# Autodesk Inventor assembly: Fr.wing_assy
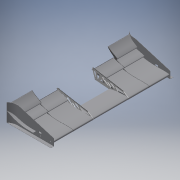
[picture p0: Inventor's stored thumbnail of the model, 180x180]
Saved by Autodesk Inventor 2018 (Build 220112000, 112)
## iProperties
Created: 2018-03-05
Part Number: Fr.wing_assy
Material: 一般
Document SubType Name: Assembly
Designer: ku_sk
Mass: 11232.8 g
Surface Area: 27769.7 cm^2
Volume: 11454.5 cm^3
Density: 0.980642 g/cm^3
Author: ku_sk
## Documents named in this file (19)
- Z:\各班フォルダ\2018\ボディ\エアロ\Aero\KS-15\Fr.wing\Fr.wing_assy.iam
- Z:\各班フォルダ\2018\ボディ\エアロ\Aero\KS-15\Fr.wing\parts\mainflap_side\mainflap_side.iam
- Z:\各班フォルダ\2018\ボディ\エアロ\Aero\KS-15\Fr.wing\parts\mainflap_center\mainflap_center.iam
- Z:\各班フォルダ\2018\ボディ\エアロ\Aero\KS-15\Fr.wing\parts\subflap\subflap.iam
- Z:\各班フォルダ\2018\ボディ\エアロ\Aero\KS-15\Fr.wing\parts\bracket1\bracket1.ipt
- Z:\各班フォルダ\2018\ボディ\エアロ\Aero\KS-15\Fr.wing\parts\bracket2.ipt
- Z:\各班フォルダ\2018\ボディ\エアロ\Aero\KS-15\Fr.wing\parts\axis_f3.ipt
- Z:\各班フォルダ\2018\ボディ\エアロ\Aero\KS-15\Fr.wing\parts\axis_f2.ipt
- Z:\各班フォルダ\2018\ボディ\エアロ\Aero\KS-15\Fr.wing\parts\axis_f1.ipt
- Z:\各班フォルダ\2018\ボディ\エアロ\Aero\KS-15\Fr.wing\parts\subflap_top.ipt
- Z:\各班フォルダ\2018\ボディ\エアロ\Aero\KS-15\Fr.wing\parts\subflap_top1.ipt
- Z:\各班フォルダ\2018\ボディ\エアロ\Aero\KS-15\Fr.wing\parts\gurnee.ipt
- Z:\各班フォルダ\2018\ボディ\エアロ\Aero\KS-15\Fr.wing\parts\gurnee_top.ipt
- Z:\各班フォルダ\2018\ボディ\エアロ\Aero\KS-15\Fr.wing\parts\endplate\ver.2\endplate_ver2.iam
- Z:\各班フォルダ\2018\ボディ\エアロ\Aero\KS-15\Fr.wing\parts\endplate\ver.2\endplate_ver21.iam
- Z:\各班フォルダ\2018\ボディ\エアロ\Aero\KS-15\Fr.wing\parts\splitter\splitter.iam
- Z:\各班フォルダ\2018\ボディ\エアロ\Aero\KS-15\Fr.wing\parts\splitter\splitter_MIR.iam
- Z:\各班フォルダ\2018\ボディ\エアロ\Aero\KS-15\Fr.wing\parts\collar_5.ipt
- Z:\各班フォルダ\2018\ボディ\エアロ\Aero\KS-15\Fr.wing\parts\collar_10.ipt
## Components (37 placed, 18 different names)
1. mainflap_center:1 [sub-assembly] — フラッシュ:1, メイト:1, メイト:4, メイト:5, メイト:6, メイト:7, 角度:1, メイト:50, メイト:51, メイト:52, メイト:53, メイト:54, メイト:55
2. mainflap_side:1 [sub-assembly] — メイト:4, メイト:7, メイト:8, メイト:9, メイト:10, フラッシュ:2, メイト:46, メイト:56, メイト:57, メイト:64
3. mainflap_side:2 [sub-assembly] — メイト:5, メイト:6, メイト:11, メイト:12, メイト:13, フラッシュ:4, メイト:49, メイト:65, メイト:93
4. mainflap_side:3 [sub-assembly] — メイト:8, メイト:9, メイト:10, フラッシュ:3, メイト:78, メイト:79, フラッシュ:20
5. mainflap_side:4 [sub-assembly] — メイト:11, メイト:12, メイト:13, フラッシュ:5
6. subflap:1 [sub-assembly] — メイト:14, メイト:15, メイト:19, フラッシュ:2, メイト:20, メイト:21, メイト:58, メイト:59
7. subflap:2 [sub-assembly] — メイト:14, メイト:15, メイト:19, フラッシュ:3
8. subflap:4 [sub-assembly] — メイト:16, メイト:17, メイト:18, フラッシュ:4, メイト:20, メイト:21, メイト:63, メイト:87, 正接:1, 正接:2
9. subflap:5 [sub-assembly] — メイト:16, メイト:17, メイト:18, フラッシュ:5, メイト:76, フラッシュ:18, メイト:77
10. bracket2:1 — メイト:46, メイト:56, メイト:57, メイト:58, メイト:59, メイト:72, メイト:73, フラッシュ:14, フラッシュ:31
11. bracket2:2 — メイト:49, メイト:63, メイト:70, メイト:71, フラッシュ:12, メイト:86, フラッシュ:28
12. bracket1:1 — メイト:52, メイト:53, メイト:54, メイト:65, メイト:88, メイト:96, メイト:97, メイト:98, メイト:99
13. bracket1:2 — メイト:50, メイト:51, メイト:55, メイト:64, メイト:74, メイト:75, フラッシュ:16, メイト:89, メイト:94, メイト:95, メイト:100, メイト:101
14. axis_f3:1 — フラッシュ:11, メイト:71, メイト:84
15. axis_f3:2 — フラッシュ:11, メイト:70, フラッシュ:12, メイト:85
16. axis_f3:3 — フラッシュ:13, メイト:73
17. axis_f3:4 — フラッシュ:13, メイト:72, フラッシュ:14
18. axis_f2:1 — フラッシュ:17, メイト:77
19. axis_f2:2 — フラッシュ:17, メイト:76, フラッシュ:18
20. axis_f2:3 — フラッシュ:15, メイト:75, フラッシュ:16
21. axis_f2:4 — フラッシュ:15, メイト:74
22. axis_f1:1 — フラッシュ:19, メイト:79
23. axis_f1:2 — フラッシュ:19, メイト:78, フラッシュ:20
24. endplate_ver2:2 [sub-assembly]
25. endplate_ver21:1 [sub-assembly]
26. subflap_top:2 — メイト:84, メイト:85, メイト:86, 正接:3, 正接:4, メイト:90
27. subflap_top1:1
28. gurnee:1 — メイト:87, 正接:1, 正接:2, メイト:88, フラッシュ:26, フラッシュ:27
29. gurnee:2 — フラッシュ:26, フラッシュ:27, メイト:89
30. gurnee_top:1 — 正接:3, 正接:4, メイト:90, フラッシュ:28, フラッシュ:29, フラッシュ:30
31. gurnee_top:2 — フラッシュ:29, フラッシュ:30, フラッシュ:31
32. splitter:2 [sub-assembly] — メイト:93
33. splitter_MIR:1 [sub-assembly]
34. collar_5:1 — メイト:94, メイト:95
35. collar_5:2 — メイト:96, メイト:97
36. collar_10:1 — メイト:98, メイト:99
37. collar_10:2 — メイト:100, メイト:101
## Relationships (86: Mate 60, Flush 21, Tangent 4, Angle 1)
- フラッシュ:1 [Flush]: mainflap_center:1
- メイト:1 [Mate]: mainflap_center:1
- メイト:4 [Mate]: mainflap_center:1 ↔ mainflap_side:1
- メイト:5 [Mate]: mainflap_center:1 ↔ mainflap_side:2
- メイト:6 [Mate]: mainflap_center:1 ↔ mainflap_side:2
- メイト:7 [Mate]: mainflap_center:1 ↔ mainflap_side:1
- メイト:8 [Mate] (4 mm): mainflap_side:1 ↔ mainflap_side:3
- メイト:9 [Mate]: mainflap_side:1 ↔ mainflap_side:3
- メイト:10 [Mate]: mainflap_side:1 ↔ mainflap_side:3
- メイト:11 [Mate] (4 mm): mainflap_side:2 ↔ mainflap_side:4
- メイト:12 [Mate]: mainflap_side:2 ↔ mainflap_side:4
- メイト:13 [Mate]: mainflap_side:2 ↔ mainflap_side:4
- メイト:14 [Mate]: subflap:1 ↔ subflap:2
- メイト:15 [Mate]: subflap:1 ↔ subflap:2
- メイト:16 [Mate] (4 mm): subflap:4 ↔ subflap:5
- メイト:17 [Mate]: subflap:4 ↔ subflap:5
- メイト:18 [Mate]: subflap:4 ↔ subflap:5
- メイト:19 [Mate] (4 mm): subflap:1 ↔ subflap:2
- フラッシュ:2 [Flush]: mainflap_side:1 ↔ subflap:1
- フラッシュ:3 [Flush]: mainflap_side:3 ↔ subflap:2
- フラッシュ:4 [Flush]: mainflap_side:2 ↔ subflap:4
- フラッシュ:5 [Flush]: mainflap_side:4 ↔ subflap:5
- メイト:20 [Mate]: subflap:1 ↔ subflap:4
- メイト:21 [Mate]: subflap:1 ↔ subflap:4
- 角度:1 [Angle] (4 deg): mainflap_center:1
- メイト:46 [Mate]: mainflap_side:1 ↔ bracket2:1
- メイト:49 [Mate]: mainflap_side:2 ↔ bracket2:2
- メイト:50 [Mate]: mainflap_center:1 ↔ bracket1:2
- メイト:51 [Mate]: mainflap_center:1 ↔ bracket1:2
- メイト:52 [Mate]: mainflap_center:1 ↔ bracket1:1
- メイト:53 [Mate]: mainflap_center:1 ↔ bracket1:1
- メイト:54 [Mate]: mainflap_center:1 ↔ bracket1:1
- メイト:55 [Mate]: mainflap_center:1 ↔ bracket1:2
- メイト:56 [Mate]: mainflap_side:1 ↔ bracket2:1
- メイト:57 [Mate]: mainflap_side:1 ↔ bracket2:1
- メイト:58 [Mate]: subflap:1 ↔ bracket2:1
- メイト:59 [Mate]: subflap:1 ↔ bracket2:1
- メイト:63 [Mate]: subflap:4 ↔ bracket2:2
- メイト:64 [Mate]: mainflap_side:1 ↔ bracket1:2
- メイト:65 [Mate]: mainflap_side:2 ↔ bracket1:1
- フラッシュ:11 [Flush]: axis_f3:1 ↔ axis_f3:2
- メイト:70 [Mate]: bracket2:2 ↔ axis_f3:2
- メイト:71 [Mate]: bracket2:2 ↔ axis_f3:1
- フラッシュ:12 [Flush]: bracket2:2 ↔ axis_f3:2
- フラッシュ:13 [Flush]: axis_f3:3 ↔ axis_f3:4
- メイト:72 [Mate]: bracket2:1 ↔ axis_f3:4
- メイト:73 [Mate]: bracket2:1 ↔ axis_f3:3
- フラッシュ:14 [Flush]: bracket2:1 ↔ axis_f3:4
- フラッシュ:15 [Flush]: axis_f2:3 ↔ axis_f2:4
- メイト:74 [Mate]: bracket1:2 ↔ axis_f2:4
- メイト:75 [Mate]: bracket1:2 ↔ axis_f2:3
- フラッシュ:16 [Flush]: bracket1:2 ↔ axis_f2:3
- フラッシュ:17 [Flush]: axis_f2:1 ↔ axis_f2:2
- メイト:76 [Mate]: subflap:5 ↔ axis_f2:2
- フラッシュ:18 [Flush]: subflap:5 ↔ axis_f2:2
- メイト:77 [Mate]: subflap:5 ↔ axis_f2:1
- フラッシュ:19 [Flush]: axis_f1:1 ↔ axis_f1:2
- メイト:78 [Mate]: mainflap_side:3 ↔ axis_f1:2
- メイト:79 [Mate]: mainflap_side:3 ↔ axis_f1:1
- フラッシュ:20 [Flush]: mainflap_side:3 ↔ axis_f1:2
- メイト:84 [Mate]: axis_f3:1 ↔ subflap_top:2
- メイト:85 [Mate]: axis_f3:2 ↔ subflap_top:2
- メイト:86 [Mate]: bracket2:2 ↔ subflap_top:2
- メイト:87 [Mate]: subflap:4 ↔ gurnee:1
- 正接:1 [Tangent]: subflap:4 ↔ gurnee:1
- 正接:2 [Tangent]: subflap:4 ↔ gurnee:1
- メイト:88 [Mate]: bracket1:1 ↔ gurnee:1
- フラッシュ:26 [Flush]: gurnee:1 ↔ gurnee:2
- フラッシュ:27 [Flush]: gurnee:1 ↔ gurnee:2
- メイト:89 [Mate]: bracket1:2 ↔ gurnee:2
- 正接:3 [Tangent]: subflap_top:2 ↔ gurnee_top:1
- 正接:4 [Tangent]: subflap_top:2 ↔ gurnee_top:1
- メイト:90 [Mate]: subflap_top:2 ↔ gurnee_top:1
- フラッシュ:28 [Flush]: bracket2:2 ↔ gurnee_top:1
- フラッシュ:29 [Flush]: gurnee_top:1 ↔ gurnee_top:2
- フラッシュ:30 [Flush]: gurnee_top:1 ↔ gurnee_top:2
- フラッシュ:31 [Flush]: bracket2:1 ↔ gurnee_top:2
- メイト:93 [Mate]: mainflap_side:2 ↔ splitter:2
- メイト:94 [Mate]: bracket1:2 ↔ collar_5:1
- メイト:95 [Mate]: bracket1:2 ↔ collar_5:1
- メイト:96 [Mate]: bracket1:1 ↔ collar_5:2
- メイト:97 [Mate]: bracket1:1 ↔ collar_5:2
- メイト:98 [Mate]: bracket1:1 ↔ collar_10:1
- メイト:99 [Mate]: bracket1:1 ↔ collar_10:1
- メイト:100 [Mate]: bracket1:2 ↔ collar_10:2
- メイト:101 [Mate]: bracket1:2 ↔ collar_10:2
